# Autodesk Inventor assembly: GP6-200
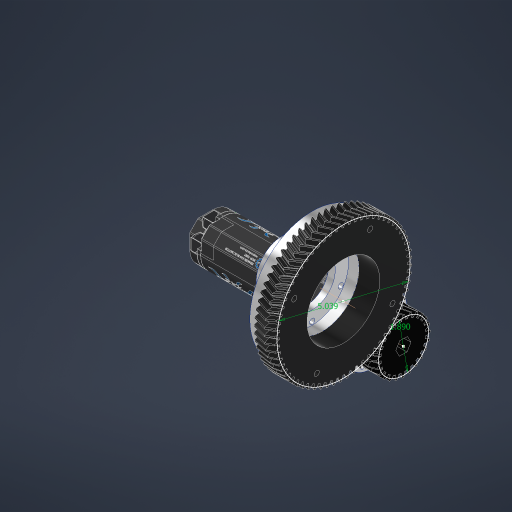
[picture p0: Inventor's stored thumbnail of the model, 512x512]
Saved by Autodesk Inventor 2023.4 (Build 274418000, 418)
## iProperties
Created: 2025-02-23
Part Number: GP6-200
Document SubType Name: Assembly
Designer: brand
Author: brand
## Documents named in this file (6)
- C:\Users\brand\OneDrive\Documents\GitHub\robotics 23\2025-ReefScape---CAD\Gripper\GP6\GP6-200.iam
- C:\Users\brand\OneDrive\Documents\GitHub\robotics 23\2025-ReefScape---CAD\Gripper\GP6\GP6-004.ipt
- C:\Users\brand\OneDrive\Documents\GitHub\robotics 23\2025-ReefScape---CAD\COMMON PARTS\4in Lazy Suzan.iam
- C:\Users\brand\OneDrive\Documents\GitHub\robotics 23\2025-ReefScape---CAD\COMMON PARTS\GEARS\Herringbone\2m 64t herringbone\2m 64t herringbone.ipt
- C:\Users\brand\OneDrive\Documents\GitHub\robotics 23\2025-ReefScape---CAD\COMMON PARTS\GEARBOXES\MAX Planetary\MAX Planetary Configurable 9-1 Kraken x44\MAX Planetary Configurable 9-1 Kraken x44.iam
- C:\Users\brand\OneDrive\Documents\GitHub\robotics 23\2025-ReefScape---CAD\COMMON PARTS\GEARS\Herringbone\herringbone 2m 24t\herringbone 2m 24t.ipt
## Components (5 placed, 5 different names)
1. GP6-004:1
2. 4in Lazy Suzan:1 [sub-assembly]
3. 2m 64t herringbone:1
4. MAX Planetary Configurable 9-1 Kraken x44:1 [sub-assembly]
5. herringbone 2m 24t:1
## Relationships (9: Insert 6, Flush 1, Tangent 1, Mate 1)
- [Insert]: GP6-004:1 ↔ 4in Lazy Suzan:1
- [Insert]: GP6-004:1 ↔ 4in Lazy Suzan:1
- [Insert]: 4in Lazy Suzan:1 ↔ 2m 64t herringbone:1
- [Insert]: 4in Lazy Suzan:1 ↔ 2m 64t herringbone:1
- [Flush]: 2m 64t herringbone:1 ↔ herringbone 2m 24t:1
- [Tangent]: 2m 64t herringbone:1 ↔ herringbone 2m 24t:1
- [Mate]: GP6-004:1 ↔ herringbone 2m 24t:1
- [Insert]: GP6-004:1 ↔ MAX Planetary Configurable 9-1 Kraken x44:1
- [Insert]: GP6-004:1 ↔ MAX Planetary Configurable 9-1 Kraken x44:1
